# Autodesk Inventor assembly: total
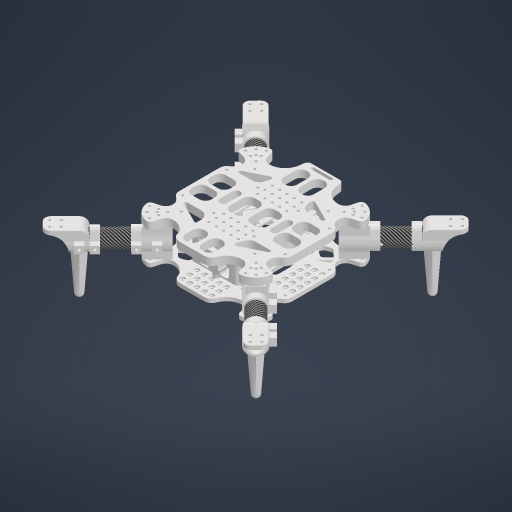
[picture p0: Inventor's stored thumbnail of the model, 512x512]
Saved by Autodesk Inventor 2023 (Build 270158000, 158)
## iProperties
Created: 2022-05-28
Part Number: total
Document SubType Name: Assembly
Designer: vibhu
Author: vibhu
## Documents named in this file (7)
- D:\Documents\_Personal\Projects\Drone\Drone\CAD\total.iam
- D:\Documents\_Personal\Projects\Drone\Drone\CAD\arm\_arm.iam
- D:\Documents\_Personal\Projects\Drone\Drone\CAD\body\bottom.ipt
- D:\Documents\_Personal\Projects\Drone\Drone\CAD\body\middle spacer bottom.ipt
- D:\Documents\_Personal\Projects\Drone\Drone\CAD\body\middle spacer top.ipt
- D:\Documents\_Personal\Projects\Drone\Drone\CAD\body\top.ipt
- D:\Documents\_Personal\Projects\Drone\Drone\CAD\body\battery holder flap.ipt
## Components (9 placed, 6 different names)
1. bottom:1 — Mate:1, Mate:2, Mate:3, Mate:4, Mate:5, Mate:6, Mate:7, Mate:8, Mate:9, Mate:10, Mate:11, Mate:12, Flush:1, Flush:3, Flush:4, Flush:5
2. _arm:1 [sub-assembly] — Mate:4, Mate:9, Mate:11
3. _arm:2 [sub-assembly] — Mate:3, Mate:7, Mate:8
4. _arm:3 [sub-assembly] — Mate:2, Mate:10, Mate:12
5. _arm:4 [sub-assembly] — Mate:1, Mate:5, Mate:6
6. middle spacer bottom:1 — Flush:1, Flush:3, Flush:4, Flush:5, Mate:13
7. middle spacer top:1 — Mate:14, Mate:15
8. top:1 — Mate:15
9. battery holder flap:1 — Mate:13, Mate:14
## Relationships (19: Mate 15, Flush 4)
- Mate:1: bottom:1 ↔ _arm:4
- Mate:2: bottom:1 ↔ _arm:3
- Mate:3: bottom:1 ↔ _arm:2
- Mate:4: bottom:1 ↔ _arm:1
- Mate:5: bottom:1 ↔ _arm:4
- Mate:6: bottom:1 ↔ _arm:4
- Mate:7: bottom:1 ↔ _arm:2
- Mate:8: bottom:1 ↔ _arm:2
- Mate:9: bottom:1 ↔ _arm:1
- Mate:10: bottom:1 ↔ _arm:3
- Mate:11: bottom:1 ↔ _arm:1
- Mate:12: bottom:1 ↔ _arm:3
- Flush:1: bottom:1 ↔ middle spacer bottom:1
- Flush:3: bottom:1 ↔ middle spacer bottom:1
- Flush:4: bottom:1 ↔ middle spacer bottom:1
- Flush:5: bottom:1 ↔ middle spacer bottom:1
- Mate:13: middle spacer bottom:1 ↔ battery holder flap:1
- Mate:14: middle spacer top:1 ↔ battery holder flap:1
- Mate:15: middle spacer top:1 ↔ top:1
